# Autodesk Inventor assembly: Payload-Interposer
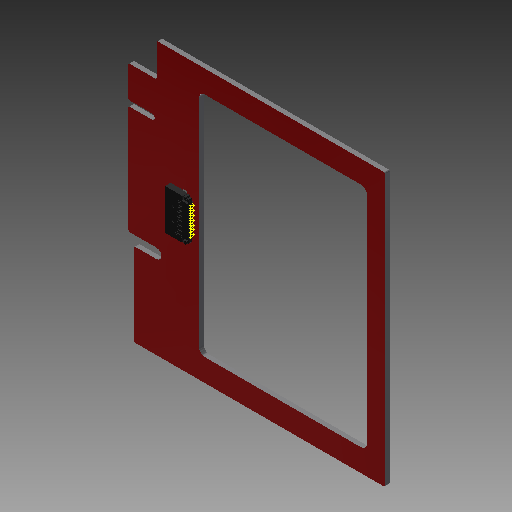
[picture p0: Inventor's stored thumbnail of the model, 512x512]
Saved by Autodesk Inventor 2018 (Build 220112000, 112)
## iProperties
Created: 2020-02-28
Part Number: Payload-Interposer
Document SubType Name: Assembly
Designer: Bradley
Author: Bradley
## Documents named in this file (3)
- C:\Users\Bradley\Documents\GitHub\CougSat1-Hardware\CougSat1-Payload\CADModel\Native\Payload-Interposer.iam
- C:\Users\Bradley\Documents\GitHub\CougSat1-Hardware\CougSat1-Payload\CADModel\Native\Payload-Interposer_PCB.ipt
- C:\Users\Bradley\Documents\GitHub\Resources\SupplierDocuments\04 - Connectors SMT\04-0007\04-0007.iam
## Components (2 placed, 2 different names)
1. Payload-Interposer_PCB:1 — Mate:1
2. 04-0007:1 [sub-assembly] — Mate:1, Mate:2, Flush:1
## Relationships (3: Mate 2, Flush 1)
- Mate:1: Payload-Interposer_PCB:1 ↔ 04-0007:1
- Mate:2: 04-0007:1
- Flush:1 (-15 mm): 04-0007:1
